# Autodesk Inventor assembly: assembly x
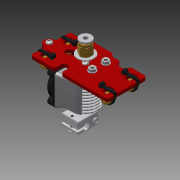
[picture p0: Inventor's stored thumbnail of the model, 180x180]
Saved by Autodesk Inventor 2015 (Build 190159000, 159)
## iProperties
Created: 2015-02-20
Part Number: assembly x
Document SubType Name: Assembly
Designer: Noa Izumi
Author: Noa Izumi
## Documents named in this file (13)
- E:\3D_Designs\Inventor\3D Printer\TinyBoy-master\src\assembly x.iam
- E:\3D_Designs\Inventor\3D Printer\TinyBoy-master\src\plastic_part_21.ipt
- E:\3D_Designs\Inventor\3D Printer\TinyBoy-master\src\plastic_part_13.ipt
- E:\3D_Designs\Inventor\3D Printer\TinyBoy-master\src\screw_M3_12_hex.ipt
- E:\3D_Designs\Inventor\3D Printer\TinyBoy-master\src\screw_M3_16_hex.ipt
- E:\3D_Designs\Inventor\3D Printer\TinyBoy-master\src\washer_M3.ipt
- E:\3D_Designs\Inventor\3D Printer\TinyBoy-master\src\ring_488.ipt
- E:\3D_Designs\Inventor\3D Printer\TinyBoy-master\src\nut_M3.ipt
- E:\3D_Designs\Inventor\3D Printer\TinyBoy-master\src\screw_M3_10_hex.ipt
- E:\3D_Designs\Inventor\3D Printer\TinyBoy-master\src\fastener_01.ipt
- E:\3D_Designs\Inventor\3D Printer\TinyBoy-master\src\plastic_part_22.ipt
- E:\3D_Designs\Inventor\3D Printer\TinyBoy-master\src\e3d_v6.iam
- E:\3D_Designs\Inventor\3D Printer\TinyBoy-master\src\bearing_603zz.ipt
## Components (27 placed, 12 different names)
1. plastic_part_21:1 — 插入:1, 插入:2, 插入:3, 插入:12, 插入:13, 插入:16, 插入:17, 插入:22, 插入:23, 角度:5, Flush:1, Mate:2, Angle:6, Mate:3, Angle:7, Mate:12, Mate:13, Mate:14, Mate:15, Mate:20, Mate:21, Mate:22, Mate:23, Mate:24, Mate:25, Mate:26, Mate:27
2. plastic_part_13:1 — 插入:2, 插入:3, 插入:4, 插入:5
3. screw_M3_12_hex:1 — 插入:1
4. screw_M3_16_hex:1 — 插入:10
5. screw_M3_16_hex:2 — 插入:11
6. bearing_603zz:1 — 插入:8, 插入:11
7. bearing_603zz:2 — 插入:9, 插入:10
8. washer_M3:1 — 插入:13, 插入:14
9. washer_M3:2 — 插入:6, 插入:8
10. washer_M3:3 — 插入:5, 插入:7
11. washer_M3:4 — 插入:4, 插入:6
12. washer_M3:5 — 插入:7, 插入:9
13. washer_M3:6 — 插入:12, 插入:15
14. ring_488:1 — Mate:8, Mate:14, Mate:18
15. ring_488:2 — Mate:9, Mate:15, Mate:16
16. ring_488:3 — Mate:11, Mate:13, Mate:19
17. ring_488:4 — Mate:10, Mate:12, Mate:17
18. nut_M3:1 — 插入:15
19. nut_M3:2 — 插入:14
20. screw_M3_10_hex:1 — 插入:17
21. screw_M3_10_hex:2 — 插入:16
22. fastener_01:1 — Mate:18, Mate:21, Mate:24
23. fastener_01:2 — Mate:17, Mate:22, Mate:27
24. fastener_01:3 — Mate:19, Mate:20, Mate:25
25. fastener_01:4 — Mate:16, Mate:23, Mate:26
26. plastic_part_22:1 — 插入:22, 插入:23, 插入:24
27. e3d_v6:1 [sub-assembly] — 插入:24, 角度:5
## Relationships (50: Mate 26, Insert 20, Angle 3, Flush 1)
- 插入:1 [Insert]: plastic_part_21:1 ↔ screw_M3_12_hex:1
- 插入:2 [Insert]: plastic_part_21:1 ↔ plastic_part_13:1
- 插入:3 [Insert]: plastic_part_21:1 ↔ plastic_part_13:1
- 插入:4 [Insert]: plastic_part_13:1 ↔ washer_M3:4
- 插入:5 [Insert]: plastic_part_13:1 ↔ washer_M3:3
- 插入:6 [Insert]: washer_M3:2 ↔ washer_M3:4
- 插入:7 [Insert]: washer_M3:3 ↔ washer_M3:5
- 插入:8 [Insert]: bearing_603zz:1 ↔ washer_M3:2
- 插入:9 [Insert]: bearing_603zz:2 ↔ washer_M3:5
- 插入:10 [Insert]: screw_M3_16_hex:1 ↔ bearing_603zz:2
- 插入:11 [Insert]: screw_M3_16_hex:2 ↔ bearing_603zz:1
- 插入:12 [Insert]: plastic_part_21:1 ↔ washer_M3:6
- 插入:13 [Insert]: plastic_part_21:1 ↔ washer_M3:1
- 插入:14 [Insert]: washer_M3:1 ↔ nut_M3:2
- 插入:15 [Insert]: washer_M3:6 ↔ nut_M3:1
- 插入:16 [Insert]: plastic_part_21:1 ↔ screw_M3_10_hex:2
- 插入:17 [Insert]: plastic_part_21:1 ↔ screw_M3_10_hex:1
- 插入:22 [Insert]: plastic_part_21:1 ↔ plastic_part_22:1
- 插入:23 [Insert]: plastic_part_21:1 ↔ plastic_part_22:1
- 插入:24 [Insert]: plastic_part_22:1 ↔ e3d_v6:1
- 角度:5 [Angle] (0 deg): plastic_part_21:1 ↔ e3d_v6:1
- Flush:1 (3 mm): plastic_part_21:1
- Mate:2: plastic_part_21:1
- Angle:6 (0 deg): plastic_part_21:1
- Mate:3: plastic_part_21:1
- Angle:7 (0 deg): plastic_part_21:1
- Mate:4
- Mate:5
- Mate:6
- Mate:7
- Mate:8: ring_488:1
- Mate:9: ring_488:2
- Mate:10: ring_488:4
- Mate:11: ring_488:3
- Mate:12: plastic_part_21:1 ↔ ring_488:4
- Mate:13: plastic_part_21:1 ↔ ring_488:3
- Mate:14: plastic_part_21:1 ↔ ring_488:1
- Mate:15: plastic_part_21:1 ↔ ring_488:2
- Mate:16: ring_488:2 ↔ fastener_01:4
- Mate:17: ring_488:4 ↔ fastener_01:2
- Mate:18: ring_488:1 ↔ fastener_01:1
- Mate:19: ring_488:3 ↔ fastener_01:3
- Mate:20: plastic_part_21:1 ↔ fastener_01:3
- Mate:21: plastic_part_21:1 ↔ fastener_01:1
- Mate:22: plastic_part_21:1 ↔ fastener_01:2
- Mate:23: plastic_part_21:1 ↔ fastener_01:4
- Mate:24: plastic_part_21:1 ↔ fastener_01:1
- Mate:25: plastic_part_21:1 ↔ fastener_01:3
- Mate:26: plastic_part_21:1 ↔ fastener_01:4
- Mate:27: plastic_part_21:1 ↔ fastener_01:2
